# Autodesk Inventor assembly: 总装配
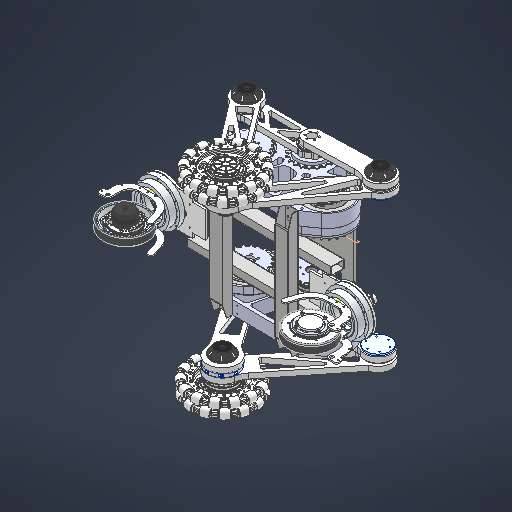
[picture p0: Inventor's stored thumbnail of the model, 512x512]
Saved by Autodesk Inventor 2025 (Build 290162000, 162)
## iProperties
Created: 2025-04-19
Part Number: 总装配
Document SubType Name: Assembly
Designer: XH
Author: XH
## Documents named in this file (7)
- C:\1A_Engineering_files\RCInventor\铝件版本\总装配.iam
- C:\1A_Engineering_files\RCInventor\铝件版本\装配体2_MIR1.iam
- C:\1A_Engineering_files\RCInventor\铝件版本\铝方管\40x15_MIR.ipt
- C:\1A_Engineering_files\RCInventor\铝件版本\轮系\舵轮\RMDL2.0——00.iam
- C:\1A_Engineering_files\RCInventor\铝件版本\碳纤维(cnc)-关节电机端子延展固定_MIR1.ipt
- C:\1A_Engineering_files\RCInventor\铝件版本\铝方管\321x30.ipt
- C:\1A_Engineering_files\RCInventor\铝件版本\板材料\玻纤\玻纤.ipt
## Components (10 placed, 6 different names)
1. 装配体2_MIR1:1 [sub-assembly] — 表面齐平:7, 表面齐平:8, 配合:10, 配合:14, 配合:15, 配合:16, 配合:22, 配合:23, 配合:24, 配合:26, 表面齐平:13
2. 40x15_MIR:1 — 表面齐平:7, 表面齐平:8, 配合:10, 配合:18, 配合:19
3. 40x15_MIR:2 — 配合:14, 配合:15, 配合:16, 配合:17, 配合:20, 配合:21, 配合:25
4. RMDL2.0——00:1 [sub-assembly] — 配合:21, 表面齐平:9, 表面齐平:10
5. 装配体2_MIR1:2 [sub-assembly] — 配合:17, 配合:18, 配合:19, 配合:20, 配合:27
6. 碳纤维(cnc)-关节电机端子延展固定_MIR1:1 — 配合:22, 配合:23, 配合:24
7. RMDL2.0——00:2 [sub-assembly] — 表面齐平:9, 表面齐平:10
8. 321x30:1 — 配合:25, 表面齐平:11, 表面齐平:12
9. 321x30:2 — 表面齐平:11, 表面齐平:12
10. 玻纤:1 — 配合:26, 表面齐平:13, 配合:27
## Relationships (23: Mate 15, Flush 8)
- 表面齐平:1 [Flush] (138 mm)
- 表面齐平:7 [Flush]: 装配体2_MIR1:1 ↔ 40x15_MIR:1
- 表面齐平:8 [Flush]: 装配体2_MIR1:1 ↔ 40x15_MIR:1
- 配合:10 [Mate]: 装配体2_MIR1:1 ↔ 40x15_MIR:1
- 配合:14 [Mate]: 装配体2_MIR1:1 ↔ 40x15_MIR:2
- 配合:15 [Mate]: 装配体2_MIR1:1 ↔ 40x15_MIR:2
- 配合:16 [Mate]: 装配体2_MIR1:1 ↔ 40x15_MIR:2
- 配合:17 [Mate]: 40x15_MIR:2 ↔ 装配体2_MIR1:2
- 配合:18 [Mate]: 40x15_MIR:1 ↔ 装配体2_MIR1:2
- 配合:19 [Mate]: 40x15_MIR:1 ↔ 装配体2_MIR1:2
- 配合:20 [Mate]: 40x15_MIR:2 ↔ 装配体2_MIR1:2
- 配合:21 [Mate] (5 mm): 40x15_MIR:2 ↔ RMDL2.0——00:1
- 配合:22 [Mate]: 装配体2_MIR1:1 ↔ 碳纤维(cnc)-关节电机端子延展固定_MIR1:1
- 配合:23 [Mate]: 装配体2_MIR1:1 ↔ 碳纤维(cnc)-关节电机端子延展固定_MIR1:1
- 配合:24 [Mate]: 装配体2_MIR1:1 ↔ 碳纤维(cnc)-关节电机端子延展固定_MIR1:1
- 表面齐平:9 [Flush]: RMDL2.0——00:1 ↔ RMDL2.0——00:2
- 表面齐平:10 [Flush]: RMDL2.0——00:1 ↔ RMDL2.0——00:2
- 配合:25 [Mate]: 40x15_MIR:2 ↔ 321x30:1
- 表面齐平:11 [Flush]: 321x30:1 ↔ 321x30:2
- 表面齐平:12 [Flush]: 321x30:1 ↔ 321x30:2
- 配合:26 [Mate]: 装配体2_MIR1:1 ↔ 玻纤:1
- 表面齐平:13 [Flush]: 装配体2_MIR1:1 ↔ 玻纤:1
- 配合:27 [Mate]: 装配体2_MIR1:2 ↔ 玻纤:1
